# Autodesk Inventor assembly: ASY PNS 1750 filter-distribution-system 1200
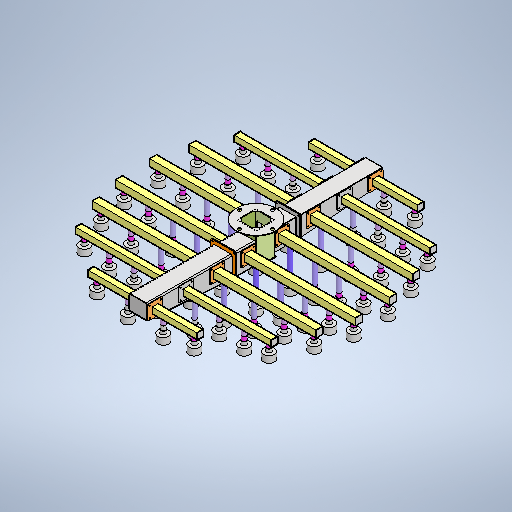
[picture p0: Inventor's stored thumbnail of the model, 512x512]
Saved by Autodesk Inventor 2025.3 (Build 293356030, 356C)
## iProperties
Created: 2025-06-24
Part Number: ASY PNS 1750 filter-distribution-system 1200
Document SubType Name: Assembly
Designer: user
Author: user
## Documents named in this file (10)
- C:\Users\admin\Yandex.Disk\home pc\Inventor\ANP--Antipayuta\ASY PNS 1750 filter-distribution-system 1200.iam
- C:\Users\admin\Yandex.Disk\home pc\Inventor\ANP--Antipayuta\Workspaces\Workspace\filter-distribution-system\PNS 1759 DIM filter-distribution-system 1200.ipt
- C:\Users\admin\Yandex.Disk\home pc\Inventor\ANP--Antipayuta\Workspaces\Workspace\filter-distribution-system\PNS 754 FDS 1200 FLANGE.ipt
- C:\Users\admin\Yandex.Disk\home pc\Inventor\ANP--Antipayuta\Workspaces\Workspace\filter-distribution-system\PNS 752 FDS 1200 FLANGE 2.ipt
- C:\Users\admin\Yandex.Disk\home pc\Inventor\ANP--Antipayuta\PNS 765 FDS 1200 CUP 1.ipt
- C:\Users\admin\Yandex.Disk\home pc\Inventor\ANP--Antipayuta\FDS 1400\ASY ANP 1490 FDS one way.iam
- C:\Users\admin\Yandex.Disk\home pc\Inventor\ANP--Antipayuta\FDS 1400\ASY ANP 1424 FDS way 4.iam
- C:\Users\admin\Yandex.Disk\home pc\Inventor\ANP--Antipayuta\Workspaces\Workspace\filter-distribution-system\PNS 753 FDS 1200 FLANGE 2 up.ipt
- C:\Users\admin\Yandex.Disk\home pc\Inventor\ANP--Antipayuta\FDS 1400\ANP 1421 FDS Diam way flange 1.ipt
- C:\Users\admin\Yandex.Disk\home pc\Inventor\ANP--Antipayuta\Workspaces\Workspace\filter-distribution-system\PNS 754 FDS 1200 FLANGE 2 down.ipt
## Components (17 placed, 14 different names)
1. PNS 1759 DIM filter-distribution-system 1200.ipt:1 — Mate:4, Mate:5
2. PNS 753 FDS 1200 FLANGE 2.ipt:1 — Mate:8, Flush:7, Flush:8, Rigid:40, Rigid:41
3. PNS 753 FDS 1200 FLANGE 2:3
4. PNS 752 FDS 1200 FLANGE 2.ipt:2 — Rigid:1, Mate:1, Flush:2, Rigid:48
5. ANP 1421 FDS Diam way flange 1:2
6. PNS 765 FDS 1200 CUP 1.ipt:1 — Mate:6, Flush:3, Flush:4
7. PNS 754 FDS 1200 FLANGE.ipt:1 — Mate:1, Flush:1, Flush:2
8. PNS 752 FDS 1200 FLANGE 2.ipt:1 — Rigid:1, Flush:1, Mate:6, Flush:3, Flush:4, Rigid:42
9. PNS 754 FDS 1200 FLANGE 2 down:2 — Rigid:48
10. PNS 754 FDS 1200 FLANGE 2 down.ipt:1 — Rigid:40, Rigid:42, Rigid:43
11. ASY ANP 1424 FDS way 4:2 [sub-assembly] — Rigid:43
12. ASY ANP 1424 FDS way 4:3 [sub-assembly]
13. ANP 1421 FDS Diam way flange 1.ipt:1 — Mate:8, Flush:7, Flush:8, Rigid:39
14. ASY ANP 1424 FDS way 4:4 [sub-assembly]
15. ASY ANP 1424 FDS way 4.iam:1 [sub-assembly] — Rigid:41
16. ASY ANP 1490 FDS one way:2 [sub-assembly]
17. ASY ANP 1490 FDS one way.iam:1 [sub-assembly] — Rigid:39
## Relationships (25: WeldJoint 11, Flush 8, Mate 6)
- Rigid:1 [WeldJoint]: PNS 752 FDS 1200 FLANGE 2.ipt:2 ↔ PNS 752 FDS 1200 FLANGE 2.ipt:1
- Mate:1: PNS 752 FDS 1200 FLANGE 2.ipt:2 ↔ PNS 754 FDS 1200 FLANGE.ipt:1
- Flush:1: PNS 754 FDS 1200 FLANGE.ipt:1 ↔ PNS 752 FDS 1200 FLANGE 2.ipt:1
- Flush:2: PNS 752 FDS 1200 FLANGE 2.ipt:2 ↔ PNS 754 FDS 1200 FLANGE.ipt:1
- Mate:4: PNS 1759 DIM filter-distribution-system 1200.ipt:1
- Mate:5: PNS 1759 DIM filter-distribution-system 1200.ipt:1
- Mate:6: PNS 765 FDS 1200 CUP 1.ipt:1 ↔ PNS 752 FDS 1200 FLANGE 2.ipt:1
- Flush:3 (-3 mm): PNS 765 FDS 1200 CUP 1.ipt:1 ↔ PNS 752 FDS 1200 FLANGE 2.ipt:1
- Flush:4 (-3 mm): PNS 765 FDS 1200 CUP 1.ipt:1 ↔ PNS 752 FDS 1200 FLANGE 2.ipt:1
- Mate:8: PNS 753 FDS 1200 FLANGE 2.ipt:1 ↔ ANP 1421 FDS Diam way flange 1.ipt:1
- Flush:7: PNS 753 FDS 1200 FLANGE 2.ipt:1 ↔ ANP 1421 FDS Diam way flange 1.ipt:1
- Flush:8: PNS 753 FDS 1200 FLANGE 2.ipt:1 ↔ ANP 1421 FDS Diam way flange 1.ipt:1
- Rigid:39 [WeldJoint]: ANP 1421 FDS Diam way flange 1.ipt:1 ↔ ASY ANP 1490 FDS one way.iam:1
- Rigid:40 [WeldJoint]: PNS 753 FDS 1200 FLANGE 2.ipt:1 ↔ PNS 754 FDS 1200 FLANGE 2 down.ipt:1
- Rigid:41 [WeldJoint]: PNS 753 FDS 1200 FLANGE 2.ipt:1 ↔ ASY ANP 1424 FDS way 4.iam:1
- Rigid:42 [WeldJoint]: PNS 752 FDS 1200 FLANGE 2.ipt:1 ↔ PNS 754 FDS 1200 FLANGE 2 down.ipt:1
- Rigid:43 [WeldJoint]: PNS 754 FDS 1200 FLANGE 2 down.ipt:1 ↔ ASY ANP 1424 FDS way 4:2
- [Mate]: PNS 753 FDS 1200 FLANGE 2:3 ↔ ANP 1421 FDS Diam way flange 1:2
- [Flush]: PNS 753 FDS 1200 FLANGE 2:3 ↔ ANP 1421 FDS Diam way flange 1:2
- [Flush]: PNS 753 FDS 1200 FLANGE 2:3 ↔ ANP 1421 FDS Diam way flange 1:2
- [WeldJoint]: ANP 1421 FDS Diam way flange 1:2 ↔ ASY ANP 1490 FDS one way:2
- [WeldJoint]: PNS 753 FDS 1200 FLANGE 2:3 ↔ PNS 754 FDS 1200 FLANGE 2 down:2
- [WeldJoint]: PNS 753 FDS 1200 FLANGE 2:3 ↔ ASY ANP 1424 FDS way 4:3
- [WeldJoint]: PNS 754 FDS 1200 FLANGE 2 down:2 ↔ ASY ANP 1424 FDS way 4:4
- Rigid:48 [WeldJoint]: PNS 752 FDS 1200 FLANGE 2.ipt:2 ↔ PNS 754 FDS 1200 FLANGE 2 down:2
## Named parameters: d211_d202 = 0 mm, d212_d203 = 0 mm, d213_d204 = 0 mm, d214_d205 = 0 mm, d215_d207 = 0 mm, d216_d208 = 0 mm, d217_d210 = 0 mm
